# Autodesk Inventor assembly: 조립품1
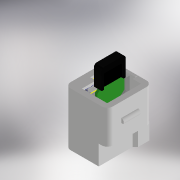
[picture p0: Inventor's stored thumbnail of the model, 180x180]
Saved by Autodesk Inventor 2020 (Build 240168000, 168)
## iProperties
Created: 2022-04-05
Part Number: 조립품1
Document SubType Name: Assembly
Designer: Knowblesse
Author: Knowblesse
## Documents named in this file (4)
- C:\VCF\Microdrive\Neuronexus\Push2Release\Neuronexus_Cap.iam
- C:\VCF\Microdrive\Neuronexus\Push2Release\CoverBody.ipt
- C:\VCF\Microdrive\Neuronexus\Push2Release\SideCover.ipt
- C:\VCF\Microdrive\Neuronexus\Neuronexus.iam
## Components (3 placed, 3 different names)
1. CoverBody:1 — 강체:1, 강체:2
2. SideCover:1 — 강체:2
3. Neuronexus:1 [sub-assembly] — 강체:1
## Relationships (2: WeldJoint 2)
- 강체:1 [WeldJoint]: CoverBody:1 ↔ Neuronexus:1
- 강체:2 [WeldJoint]: CoverBody:1 ↔ SideCover:1
